# Autodesk Inventor assembly: arm bearing support
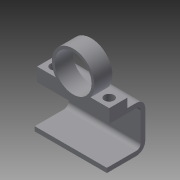
[picture p0: Inventor's stored thumbnail of the model, 180x180]
Saved by Autodesk Inventor 2013 (Build 170138000, 138)
## iProperties
Created: 2013-02-02
Part Number: arm bearing support
Document SubType Name: Assembly
Designer: aslane
Author: aslane
## Documents named in this file (3)
- \\NNHSSRV2.hs.sd203.org\aslane$\arm bearing support.iam
- \\NNHSSRV2.hs.sd203.org\aslane$\Pillow block for arm bearing.ipt
- \\NNHSSRV2.hs.sd203.org\aslane$\new support for PG-71.ipt
## Components (2 placed, 2 different names)
1. Pillow block for arm bearing:1 — Mate:1, Mate:2, Mate:3
2. new support for PG-71:1 — Mate:1, Mate:2, Mate:3
## Relationships (3: Mate 3)
- Mate:1: Pillow block for arm bearing:1 ↔ new support for PG-71:1
- Mate:2: Pillow block for arm bearing:1 ↔ new support for PG-71:1
- Mate:3: Pillow block for arm bearing:1 ↔ new support for PG-71:1
